# Autodesk Inventor assembly: 6GT28122EA01_001_STEP
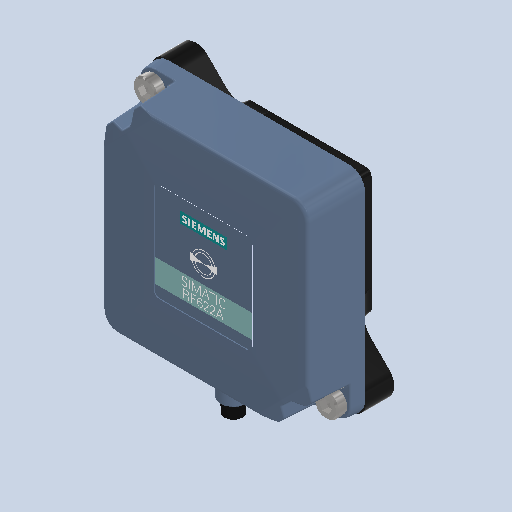
[picture p0: Inventor's stored thumbnail of the model, 512x512]
Saved by Autodesk Inventor 2023 (Build 270158000, 158)
## iProperties
Created: 2020-09-15
Part Number: 6GT28122EA01_001_STEP
Description: STEP AP214
Document SubType Name: Assembly
Designer: chriboehm
Mass: 159.253 g
Surface Area: 300.301 cm^2
Volume: 150.343 cm^3
Density: 1.05927 g/cm^3
Sending System: SolidWorks 2019
Preprocessor: SwSTEP 2.0
Title: 6GT28122EA01_001_STEP.STEP
Revision Number: ANY
## Documents named in this file (5)
- C:\work\robots\butler_2.0\body_model\parts\Reader\RF622A.iam
- C:\work\robots\butler_2.0\body_model\parts\Reader\Print_IMP.ipt
- C:\work\robots\butler_2.0\body_model\parts\Reader\Body_Normal.ipt
- C:\work\robots\butler_2.0\body_model\parts\Reader\mount.ipt
- C:\Users\chriboehm\Documents\Inventor\Content Center Files\R2023\en-US\DIN 6912\DIN 6912 - M5 x 16.ipt
## Components (5 placed, 4 different names)
1. Print_IMP_1 — Mate:5, Mate:6, Mate:7
2. Body_Normal_2 — Flush:1, Flush:2, Mate:1, Mate:2, Mate:3, Mate:4, Mate:5, Mate:6, Mate:7
3. mount:1 — Flush:1, Flush:2
4. DIN 6912 M5 x 16:1 — Mate:1, Mate:2
5. DIN 6912 M5 x 16:2 — Mate:3, Mate:4
## Relationships (9: Mate 7, Flush 2)
- Flush:1: Body_Normal_2 ↔ mount:1
- Flush:2: Body_Normal_2 ↔ mount:1
- Mate:1: Body_Normal_2 ↔ DIN 6912 M5 x 16:1
- Mate:2: Body_Normal_2 ↔ DIN 6912 M5 x 16:1
- Mate:3: Body_Normal_2 ↔ DIN 6912 M5 x 16:2
- Mate:4: Body_Normal_2 ↔ DIN 6912 M5 x 16:2
- Mate:5: Print_IMP_1 ↔ Body_Normal_2
- Mate:6 (0.25 mm): Print_IMP_1 ↔ Body_Normal_2
- Mate:7 (0.25 mm): Print_IMP_1 ↔ Body_Normal_2
